# Autodesk Inventor assembly: 3p-1
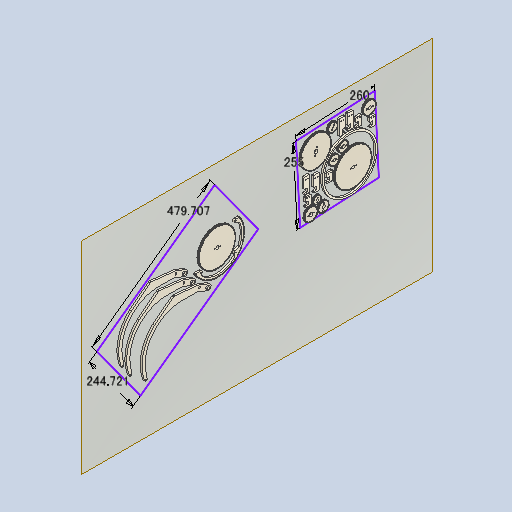
[picture p0: Inventor's stored thumbnail of the model, 512x512]
Saved by Autodesk Inventor 2025.2 (Build 292293000, 293)
## iProperties
Created: 2025-01-15
Part Number: 3p-1
Document SubType Name: Assembly
Designer: haruy
Author: haruy
## Documents named in this file (12)
- C:\Users\haruy\Documents\ロボコン\NHK2025\cad\mdf\3p-1.iam
- C:\Users\haruy\Documents\ロボコン\NHK2025\cad\nagahisa\base_weel\000-base_wheel-v1\デザイン アクセラレータ\平歯車1.iam
- C:\Users\haruy\Documents\ロボコン\NHK2025\cad\nagahisa\belt_liner\000-belt_liner_v2\デザイン アクセラレータ\平歯車1.iam
- C:\Users\haruy\Documents\ロボコン\NHK2025\cad\nagahisa\belt_liner\000-belt_liner_v1\デザイン アクセラレータ\平歯車3.iam
- C:\Users\haruy\Documents\ロボコン\NHK2025\cad\nagahisa\belt_liner\000-belt_liner_v2\デザイン アクセラレータ\平歯車2.iam
- C:\Users\haruy\Documents\ロボコン\NHK2025\cad\nagahisa\dribl\000-dribl-v1\デザイン アクセラレータ\平歯車1.iam
- C:\Users\haruy\Documents\ロボコン\NHK2025\cad\nagahisa\dribl\000-dribl-v1\デザイン アクセラレータ\平歯車2.iam
- C:\Users\haruy\Documents\ロボコン\NHK2025\cad\nagahisa\dribl\000-dribl-v1\デザイン アクセラレータ\平歯車3.iam
- C:\Users\haruy\Documents\ロボコン\NHK2025\cad\nagahisa\belt_liner\belt_liner_v2_Pom_r.ipt
- C:\Users\haruy\Documents\ロボコン\NHK2025\cad\nagahisa\hand\grab\hand-grab-v1-MDF-arm.ipt
- C:\Users\haruy\Documents\ロボコン\NHK2025\cad\nagahisa\base_weel\base_weel-v2-POM-pc-F-2.ipt
- C:\Users\haruy\Documents\ロボコン\NHK2025\cad\nagahisa\base_weel\base_weel-v2-POM-pc-F-1.ipt
## Components (20 placed, 5 different names)
1. 平歯車:1 [sub-assembly] — フラッシュ:1
2. 平歯車:2 [sub-assembly] — フラッシュ:2
3. 平歯車:3 [sub-assembly] — フラッシュ:3
4. 平歯車:4 [sub-assembly] — フラッシュ:4
5. 平歯車:5 [sub-assembly] — フラッシュ:5
6. 平歯車:6 [sub-assembly] — フラッシュ:6
7. 平歯車:7 [sub-assembly] — フラッシュ:7
8. 平歯車:8 [sub-assembly] — フラッシュ:8
9. belt_liner_v2_Pom_r:1 — フラッシュ:9
10. hand-grab-v1-MDF-arm:1 — フラッシュ:10
11. hand-grab-v1-MDF-arm:2 — フラッシュ:11
12. hand-grab-v1-MDF-arm:3 — フラッシュ:12
13. base_weel-v2-POM-pc-F-2:1 — フラッシュ:13
14. base_weel-v2-POM-pc-F-2:2 — フラッシュ:14
15. base_weel-v2-POM-pc-F-2:3 — フラッシュ:15
16. base_weel-v2-POM-pc-F-2:4 — フラッシュ:16
17. base_weel-v2-POM-pc-F-1:1 — フラッシュ:17
18. base_weel-v2-POM-pc-F-1:2 — フラッシュ:20
19. base_weel-v2-POM-pc-F-1:3 — フラッシュ:19
20. base_weel-v2-POM-pc-F-1:4 — フラッシュ:18
## Relationships (20: Flush 20)
- フラッシュ:1 [Flush]: 平歯車:1
- フラッシュ:2 [Flush]: 平歯車:2
- フラッシュ:3 [Flush]: 平歯車:3
- フラッシュ:4 [Flush]: 平歯車:4
- フラッシュ:5 [Flush]: 平歯車:5
- フラッシュ:6 [Flush]: 平歯車:6
- フラッシュ:7 [Flush]: 平歯車:7
- フラッシュ:8 [Flush]: 平歯車:8
- フラッシュ:9 [Flush]: belt_liner_v2_Pom_r:1
- フラッシュ:10 [Flush]: hand-grab-v1-MDF-arm:1
- フラッシュ:11 [Flush]: hand-grab-v1-MDF-arm:2
- フラッシュ:12 [Flush]: hand-grab-v1-MDF-arm:3
- フラッシュ:13 [Flush]: base_weel-v2-POM-pc-F-2:1
- フラッシュ:14 [Flush]: base_weel-v2-POM-pc-F-2:2
- フラッシュ:15 [Flush]: base_weel-v2-POM-pc-F-2:3
- フラッシュ:16 [Flush]: base_weel-v2-POM-pc-F-2:4
- フラッシュ:17 [Flush]: base_weel-v2-POM-pc-F-1:1
- フラッシュ:18 [Flush]: base_weel-v2-POM-pc-F-1:4
- フラッシュ:19 [Flush]: base_weel-v2-POM-pc-F-1:3
- フラッシュ:20 [Flush]: base_weel-v2-POM-pc-F-1:2
